# Autodesk Inventor assembly: FT7635M_Servo assembly
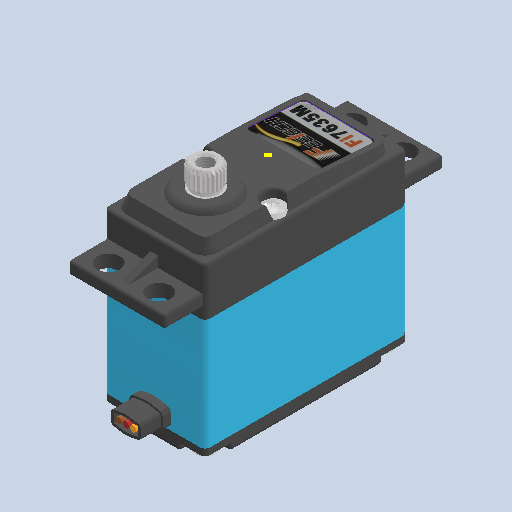
[picture p0: Inventor's stored thumbnail of the model, 512x512]
Saved by Autodesk Inventor 2025.3 (Build 293356000, 356)
## iProperties
Created: 2024-02-18
Part Number: FT7635M_Servo assembly
Document SubType Name: Assembly
Designer: Eryk
Author: Eryk
## Documents named in this file (4)
- D:\Shooting Mechanism CAD\FT7635M_Servo assembly.iam
- D:\Shooting Mechanism CAD\Body.ipt
- D:\Shooting Mechanism CAD\622162x20.ipt
- D:\Shooting Mechanism CAD\Multiple_spline_mount.ipt
## Components (8 placed, 3 different names)
1. Body:1 — Rigid:1, Rigid:2, Rigid:3, Rigid:4, Rigid:5, Rigid:6, Rotational:1
2. 622162x20:1 — Rigid:1
3. 622162x20:2 — Rigid:2
4. 622162x20:3 — Rigid:3
5. 622162x20:4 — Rigid:4
6. 622162x20:5 — Rigid:6
7. 622162x20:6 — Rigid:5
8. Multiple_spline_mount:1 — Rotational:1
## Relationships (7: WeldJoint 6, RevoluteJoint 1)
- Rigid:1 [WeldJoint]: Body:1 ↔ 622162x20:1
- Rigid:2 [WeldJoint]: Body:1 ↔ 622162x20:2
- Rigid:3 [WeldJoint]: Body:1 ↔ 622162x20:3
- Rigid:4 [WeldJoint]: Body:1 ↔ 622162x20:4
- Rigid:5 [WeldJoint]: Body:1 ↔ 622162x20:6
- Rigid:6 [WeldJoint]: Body:1 ↔ 622162x20:5
- Rotational:1 [RevoluteJoint]: Body:1 ↔ Multiple_spline_mount:1
